# Autodesk Inventor assembly: TOWER PRO MG-995, ANALOG SERVO
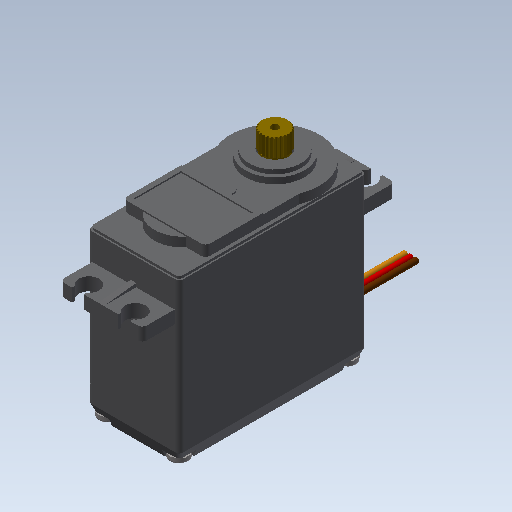
[picture p0: Inventor's stored thumbnail of the model, 512x512]
Saved by Autodesk Inventor 2020.3 (Build 243373000, 373)
## iProperties
Created: 2014-12-03
Part Number: TOWER PRO MG-995, ANALOG SERVO
Description: STEP AP214
Document SubType Name: Assembly
Designer: Nanjar
Sending System: SolidWorks 2014
Preprocessor: SwSTEP 2.0
Title: TOWER PRO MG-995, ANALOG SERVO.STEP
Revision Number: ANY
## Documents named in this file (7)
- C:\Users\Public\D\Desktop\robotic-arm-with-sensor-1.snapshot.1\Autodesk Inventor\TOWER PRO MG-995, ANALOG SERVO.iam
- C:\Users\Public\D\Desktop\robotic-arm-with-sensor-1.snapshot.1\Autodesk Inventor\TOWER PRO MG-995, ANALOG SERVO, BODY, BOTTOM.ipt
- C:\Users\Public\D\Desktop\robotic-arm-with-sensor-1.snapshot.1\Autodesk Inventor\TOWER PRO MG-995, ANALOG SERVO, BODY, MIDDLE.ipt
- C:\Users\Public\D\Desktop\robotic-arm-with-sensor-1.snapshot.1\Autodesk Inventor\TOWER PRO MG-995, ANALOG SERVO, BODY, TOP.ipt
- C:\Users\Public\D\Desktop\robotic-arm-with-sensor-1.snapshot.1\Autodesk Inventor\TOWER PRO MG-995, ANALOG SERVO, CONNECTOR.ipt
- C:\Users\Public\D\Desktop\robotic-arm-with-sensor-1.snapshot.1\Autodesk Inventor\TOWER PRO MG-995, ANALOG SERVO, SHAFT.ipt
- C:\Users\Public\D\Desktop\robotic-arm-with-sensor-1.snapshot.1\Autodesk Inventor\pan cross head_am_B18.6.7M - M2 x 0.4 x 10 Type I Cross Recessed PHMS --10N.ipt
## Components (9 placed, 9 different names)
1. TOWER PRO MG-995, ANALOG SERVO, BODY, BOTTOM_1 — Mate:1, Mate:2, Mate:3, Mate:4, Mate:5, Mate:6, Mate:7, Mate:8, Mate:9, Flush:1, Flush:2
2. TOWER PRO MG-995, ANALOG SERVO, BODY, MIDDLE_2 — Mate:9, Flush:1, Flush:2, Mate:10, Flush:3, Flush:4
3. TOWER PRO MG-995, ANALOG SERVO, BODY, TOP_3 — Mate:10, Flush:3, Flush:4, Mate:13, Flush:5
4. TOWER PRO MG-995, ANALOG SERVO, CONNECTOR_4
5. TOWER PRO MG-995, ANALOG SERVO, SHAFT_5 — Mate:13, Flush:5
6. pan cross head_am_B18.6.7M - M2 x 0.4 x 10 Type I Cross Recessed PHMS --10N_7 — Mate:3, Mate:7
7. pan cross head_am_B18.6.7M - M2 x 0.4 x 10 Type I Cross Recessed PHMS --10N_8 — Mate:2, Mate:8
8. pan cross head_am_B18.6.7M - M2 x 0.4 x 10 Type I Cross Recessed PHMS --10N_9 — Mate:1, Mate:5
9. pan cross head_am_B18.6.7M - M2 x 0.4 x 10 Type I Cross Recessed PHMS --10N_10 — Mate:4, Mate:6
## Relationships (16: Mate 11, Flush 5)
- Mate:1: TOWER PRO MG-995, ANALOG SERVO, BODY, BOTTOM_1 ↔ pan cross head_am_B18.6.7M - M2 x 0.4 x 10 Type I Cross Recessed PHMS --10N_9
- Mate:2: TOWER PRO MG-995, ANALOG SERVO, BODY, BOTTOM_1 ↔ pan cross head_am_B18.6.7M - M2 x 0.4 x 10 Type I Cross Recessed PHMS --10N_8
- Mate:3: TOWER PRO MG-995, ANALOG SERVO, BODY, BOTTOM_1 ↔ pan cross head_am_B18.6.7M - M2 x 0.4 x 10 Type I Cross Recessed PHMS --10N_7
- Mate:4: TOWER PRO MG-995, ANALOG SERVO, BODY, BOTTOM_1 ↔ pan cross head_am_B18.6.7M - M2 x 0.4 x 10 Type I Cross Recessed PHMS --10N_10
- Mate:5: TOWER PRO MG-995, ANALOG SERVO, BODY, BOTTOM_1 ↔ pan cross head_am_B18.6.7M - M2 x 0.4 x 10 Type I Cross Recessed PHMS --10N_9
- Mate:6: TOWER PRO MG-995, ANALOG SERVO, BODY, BOTTOM_1 ↔ pan cross head_am_B18.6.7M - M2 x 0.4 x 10 Type I Cross Recessed PHMS --10N_10
- Mate:7: TOWER PRO MG-995, ANALOG SERVO, BODY, BOTTOM_1 ↔ pan cross head_am_B18.6.7M - M2 x 0.4 x 10 Type I Cross Recessed PHMS --10N_7
- Mate:8: TOWER PRO MG-995, ANALOG SERVO, BODY, BOTTOM_1 ↔ pan cross head_am_B18.6.7M - M2 x 0.4 x 10 Type I Cross Recessed PHMS --10N_8
- Mate:9: TOWER PRO MG-995, ANALOG SERVO, BODY, BOTTOM_1 ↔ TOWER PRO MG-995, ANALOG SERVO, BODY, MIDDLE_2
- Flush:1: TOWER PRO MG-995, ANALOG SERVO, BODY, BOTTOM_1 ↔ TOWER PRO MG-995, ANALOG SERVO, BODY, MIDDLE_2
- Flush:2: TOWER PRO MG-995, ANALOG SERVO, BODY, BOTTOM_1 ↔ TOWER PRO MG-995, ANALOG SERVO, BODY, MIDDLE_2
- Mate:10: TOWER PRO MG-995, ANALOG SERVO, BODY, MIDDLE_2 ↔ TOWER PRO MG-995, ANALOG SERVO, BODY, TOP_3
- Flush:3: TOWER PRO MG-995, ANALOG SERVO, BODY, MIDDLE_2 ↔ TOWER PRO MG-995, ANALOG SERVO, BODY, TOP_3
- Flush:4: TOWER PRO MG-995, ANALOG SERVO, BODY, MIDDLE_2 ↔ TOWER PRO MG-995, ANALOG SERVO, BODY, TOP_3
- Mate:13: TOWER PRO MG-995, ANALOG SERVO, BODY, TOP_3 ↔ TOWER PRO MG-995, ANALOG SERVO, SHAFT_5
- Flush:5: TOWER PRO MG-995, ANALOG SERVO, BODY, TOP_3 ↔ TOWER PRO MG-995, ANALOG SERVO, SHAFT_5
